# Autodesk Inventor assembly: Oring_KF_part
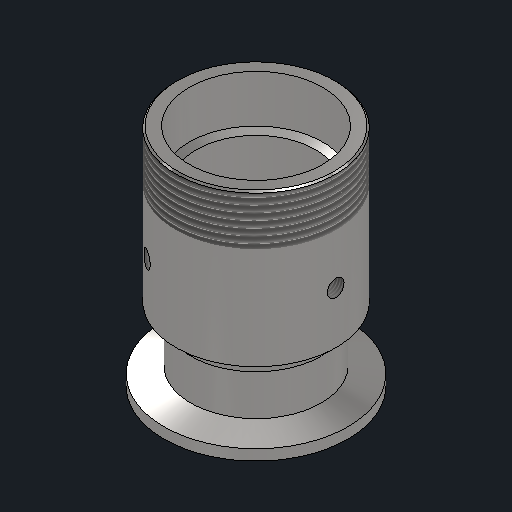
[picture p0: Inventor's stored thumbnail of the model, 512x512]
Saved by Autodesk Inventor 2026 (Build 300175050, 175E)
## iProperties
Created: 2022-12-02
Part Number: Oring_KF_part
Document SubType Name: Assembly
Designer: kuzmin
Author: kuzmin
## Documents named in this file (3)
- C:\Users\queez\Dropbox\Drawings\PIHTI\PALP\Oring-seal\Oring_KF_part.iam
- C:\Users\queez\Dropbox\Drawings\PIHTI\PALP\Oring-seal\OringNut.ipt
- C:\Users\queez\Dropbox\Drawings\PIHTI\PALP\Oring-seal\KF40_welding_part.ipt
## Components (2 placed, 2 different names)
1. OringNut:1 — Mate:1, Mate:2, Mate:3, Rotational:1
2. KF40_welding_part:1 — Rotational:1
## Relationships (4: Mate 3, RevoluteJoint 1)
- Mate:1: OringNut:1
- Mate:2: OringNut:1
- Mate:3: OringNut:1
- Rotational:1 [RevoluteJoint]: OringNut:1 ↔ KF40_welding_part:1
